# Autodesk Inventor assembly: Ricea f. Florentina alexandra-T6
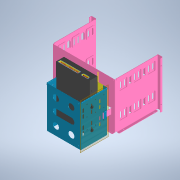
[picture p0: Inventor's stored thumbnail of the model, 180x180]
Saved by Autodesk Inventor 2022 (Build 260153000, 153)
## iProperties
Created: 2022-02-22
Part Number: Ricea f. Florentina alexandra-T6
Document SubType Name: Assembly
Designer: mtrot
Student_ACE: Necsulea i. M. Adrian stefanita
Grupa_ACE: CR-1.2.b
Tema_ACE: 6-Ansamblu suporti table
An_ACE: 2022
Author: mtrot
## Documents named in this file (6)
- C:\Users\Alexandra\Desktop\Tema6\Ricea f. Florentina alexandra-T6.iam
- C:\Users\Alexandra\Desktop\Tema6\Ricea f. Florentina alexandra-T5_SuportHdd.ipt
- C:\Users\Alexandra\Desktop\Tema6\CapacSuport.ipt
- C:\Users\Alexandra\Desktop\Tema6\SuportCD.ipt
- C:\Users\Alexandra\Desktop\Tema6\Hdd.ipt
- C:\Users\Alexandra\Documents\Inventor\Content Center Files\R2022\en-US\ISO 7045  H\ISO 7045 - M4 x 5_ - 4.8 - H - ISO.ipt
## Components (8 placed, 5 different names)
1. Ricea f. Florentina alexandra-T5_SuportHdd:1 — Flush:1, Flush:2, Flush:3, Flush:4, Mate:3, Mate:4, Angle:1, Mate:6, Mate:8
2. CapacSuport:1 — Flush:1, Flush:2, Mate:1, Mate:2
3. SuportCD:1 — Mate:1, Mate:2, Flush:3, Flush:4
4. Hdd:1 — Mate:3, Mate:4, Angle:1, Mate:5, Mate:7, Mate:11, Mate:12, Mate:13, Mate:14
5. ISO 7045 H M4 x 5 - 4.8 - H:1 — Mate:5, Mate:6
6. ISO 7045 H M4 x 5 - 4.8 - H:2 — Mate:7, Mate:8
7. ISO 7045 H M4 x 5 - 4.8 - H:4 — Mate:11, Mate:12
8. ISO 7045 H M4 x 5 - 4.8 - H:5 — Mate:13, Mate:14
## Relationships (17: Mate 12, Flush 4, Angle 1)
- Flush:1: Ricea f. Florentina alexandra-T5_SuportHdd:1 ↔ CapacSuport:1
- Flush:2: Ricea f. Florentina alexandra-T5_SuportHdd:1 ↔ CapacSuport:1
- Mate:1: CapacSuport:1 ↔ SuportCD:1
- Mate:2: CapacSuport:1 ↔ SuportCD:1
- Flush:3 (11 mm): Ricea f. Florentina alexandra-T5_SuportHdd:1 ↔ SuportCD:1
- Flush:4: Ricea f. Florentina alexandra-T5_SuportHdd:1 ↔ SuportCD:1
- Mate:3: Ricea f. Florentina alexandra-T5_SuportHdd:1 ↔ Hdd:1
- Mate:4: Ricea f. Florentina alexandra-T5_SuportHdd:1 ↔ Hdd:1
- Angle:1 (0 deg): Ricea f. Florentina alexandra-T5_SuportHdd:1 ↔ Hdd:1
- Mate:5: Hdd:1 ↔ ISO 7045 H M4 x 5 - 4.8 - H:1
- Mate:6: Ricea f. Florentina alexandra-T5_SuportHdd:1 ↔ ISO 7045 H M4 x 5 - 4.8 - H:1
- Mate:7: Hdd:1 ↔ ISO 7045 H M4 x 5 - 4.8 - H:2
- Mate:8: Ricea f. Florentina alexandra-T5_SuportHdd:1 ↔ ISO 7045 H M4 x 5 - 4.8 - H:2
- Mate:11: Hdd:1 ↔ ISO 7045 H M4 x 5 - 4.8 - H:4
- Mate:12: Hdd:1 ↔ ISO 7045 H M4 x 5 - 4.8 - H:4
- Mate:13: Hdd:1 ↔ ISO 7045 H M4 x 5 - 4.8 - H:5
- Mate:14: Hdd:1 ↔ ISO 7045 H M4 x 5 - 4.8 - H:5
